# Autodesk Inventor assembly: NewTail(final)
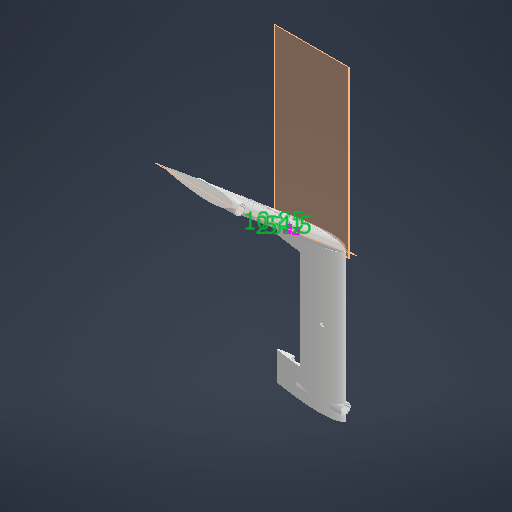
[picture p0: Inventor's stored thumbnail of the model, 512x512]
Saved by Autodesk Inventor 2026 (Build 300175050, 175E)
## iProperties
Created: 2026-08-04
Part Number: NewTail(final)
Document SubType Name: Assembly
Designer: Delbe
Author: Delbe
## Documents named in this file (3)
- C:\GitHub\SWIFT-UAV\System_development\Pelican\structural_model\v0.3.0\Parts\Delb_Parts\NewTail(final).iam
- C:\GitHub\SWIFT-UAV\System_development\Pelican\structural_model\v0.3.0\Parts\Delb_Parts\Delb_Tail_Male(fr).iam
- C:\GitHub\SWIFT-UAV\System_development\Pelican\structural_model\v0.3.0\Parts\Delb_Parts\Female_Tail_v2.iam
## Components (2 placed, 2 different names)
1. Delb_Tail_Male(fr):1 [sub-assembly] — Rigid:1
2. Female_Tail_v2:1 [sub-assembly] — Rigid:1
## Relationships (1: WeldJoint 1)
- Rigid:1 [WeldJoint]: Delb_Tail_Male(fr):1 ↔ Female_Tail_v2:1
